# Autodesk Inventor assembly: Assembly1
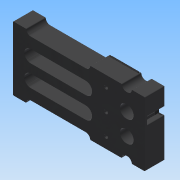
[picture p0: Inventor's stored thumbnail of the model, 180x180]
Saved by Autodesk Inventor 2016 (Build 200138000, 138)
## iProperties
Created: 2015-08-28
Part Number: Assembly1
Document SubType Name: Assembly
Designer: Openlab
Author: Openlab
## Documents named in this file (3)
- D:\Alexey\HS-Spectrophotometer\parts\Paris\Assembly1.iam
- D:\Alexey\HS-Spectrophotometer\parts\Paris\Core_bottom-im.ipt
- D:\Alexey\HS-Spectrophotometer\parts\Paris\Core_top-im.ipt
## Components (2 placed, 2 different names)
1. Core_bottom-im:1 — Mate:1, Mate:2, Mate:3
2. Core_top-im:1 — Mate:1, Mate:2, Mate:3
## Relationships (3: Mate 3)
- Mate:1: Core_bottom-im:1 ↔ Core_top-im:1
- Mate:2: Core_bottom-im:1 ↔ Core_top-im:1
- Mate:3: Core_bottom-im:1 ↔ Core_top-im:1
